# Autodesk Inventor assembly: КВ33.044.900 - Клапан присоски впускной
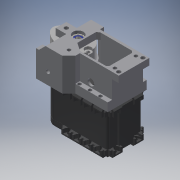
[picture p0: Inventor's stored thumbnail of the model, 180x180]
Saved by Autodesk Inventor 2019 (Build 230136000, 136)
## iProperties
Created: 2019-08-25
Part Number: КВ33.044.900 - Клапан присоски впускной
Material: Типовые
Document SubType Name: Assembly
Designer: Петров Иван
Author: Петров Иван
## Documents named in this file (6)
- E:\IVAN\Kvantoriada2019\optimal_gripper\hardware\КВ33.044.900 - Клапан присоски впускной.iam
- E:\IVAN\Kvantoriada2019\optimal_gripper\hardware\КВ33.044.901  - Опора клапана присоски.ipt
- E:\IVAN\Kvantoriada2019\optimal_gripper\hardware\Стандартные изделия\Сервомотор Dynamixel AX-12A\ax-12a.iam
- E:\IVAN\Kvantoriada2019\optimal_gripper\hardware\Стандартные изделия\Проставка 5.5 мм.ipt
- E:\IVAN\Kvantoriada2019\optimal_gripper\hardware\КВ33.044.902 - Кулачок дисковый.ipt
- E:\IVAN\Kvantoriada2019\optimal_gripper\hardware\Стандартные изделия\Подшипник 4x8x3.ipt
## Components (5 placed, 5 different names)
1. КВ33.044.901  - Опора клапана присоски:1 — Совмещение:1, Совмещение:2, Совмещение:3, Заподлицо:1, Совмещение:9
2. ax-12a:1 [sub-assembly] — Совмещение:1, Совмещение:2, Совмещение:3, Совмещение:4, Совмещение:5
3. Проставка 5.5 мм:1 — Совмещение:4, Совмещение:5, Совмещение:6, Совмещение:7, Совмещение:8
4. Дисковый кулачок:1 — Совмещение:6, Совмещение:7, Совмещение:8
5. Подшипник 4x8x3:1 — Заподлицо:1, Совмещение:9
## Relationships (10: Mate 9, Flush 1)
- Совмещение:1 [Mate]: КВ33.044.901  - Опора клапана присоски:1 ↔ ax-12a:1
- Совмещение:2 [Mate]: КВ33.044.901  - Опора клапана присоски:1 ↔ ax-12a:1
- Совмещение:3 [Mate]: КВ33.044.901  - Опора клапана присоски:1 ↔ ax-12a:1
- Совмещение:4 [Mate]: ax-12a:1 ↔ Проставка 5.5 мм:1
- Совмещение:5 [Mate]: ax-12a:1 ↔ Проставка 5.5 мм:1
- Совмещение:6 [Mate]: Проставка 5.5 мм:1 ↔ Дисковый кулачок:1
- Совмещение:7 [Mate]: Проставка 5.5 мм:1 ↔ Дисковый кулачок:1
- Совмещение:8 [Mate]: Проставка 5.5 мм:1 ↔ Дисковый кулачок:1
- Заподлицо:1 [Flush]: КВ33.044.901  - Опора клапана присоски:1 ↔ Подшипник 4x8x3:1
- Совмещение:9 [Mate]: КВ33.044.901  - Опора клапана присоски:1 ↔ Подшипник 4x8x3:1
